# Autodesk Inventor assembly: Assy_linear_module
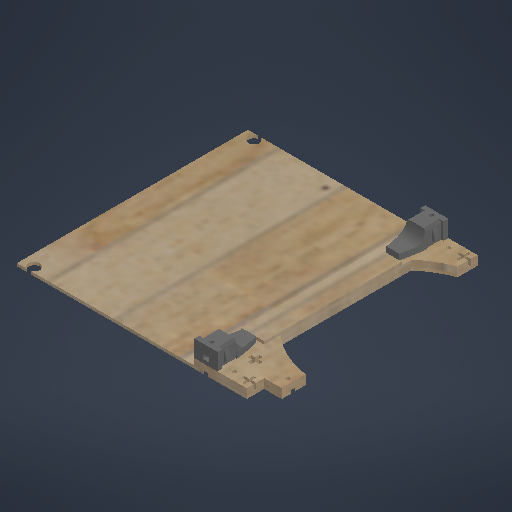
[picture p0: Inventor's stored thumbnail of the model, 512x512]
Saved by Autodesk Inventor 2026.1 (Build 301233020, 233B)
## iProperties
Created: 2025-09-27
Part Number: Assy_linear_module
Document SubType Name: Assembly
Designer: hibik
Author: hibik
## Documents named in this file (5)
- C:\Users\hibik\Documents\Robomech\conveyer\liniar_module\Assy_linear_module.iam
- C:\Users\hibik\Documents\Robomech\conveyer\liniar_module\base.ipt
- C:\Users\hibik\Documents\Robomech\conveyer\liniar_module\connector_base.ipt
- C:\Users\hibik\Documents\Robomech\conveyer\liniar_module\back_upper.ipt
- C:\Users\hibik\Documents\Robomech\conveyer\connector_module\connector_male.ipt
## Components (5 placed, 4 different names)
1. base:1 — メイト:1, フラッシュ:1, フラッシュ:2, フラッシュ:3, フラッシュ:4
2. connector_base:1 — メイト:1, メイト:2, フラッシュ:1, フラッシュ:3, 挿入:2, 角度:3, 挿入:5, 角度:4
3. back_upper:1 — メイト:2, フラッシュ:2, フラッシュ:4
4. connector_male:4 — 挿入:2, 角度:3
5. connector_male:6 — 挿入:5, 角度:4
## Relationships (10: Flush 4, Mate 2, Insert 2, Angle 2)
- メイト:1 [Mate]: base:1 ↔ connector_base:1
- メイト:2 [Mate]: connector_base:1 ↔ back_upper:1
- フラッシュ:1 [Flush]: base:1 ↔ connector_base:1
- フラッシュ:2 [Flush]: base:1 ↔ back_upper:1
- フラッシュ:3 [Flush]: base:1 ↔ connector_base:1
- フラッシュ:4 [Flush]: base:1 ↔ back_upper:1
- 挿入:2 [Insert]: connector_base:1 ↔ connector_male:4
- 角度:3 [Angle] (0 deg): connector_base:1 ↔ connector_male:4
- 挿入:5 [Insert]: connector_base:1 ↔ connector_male:6
- 角度:4 [Angle] (0 deg): connector_base:1 ↔ connector_male:6
